# Autodesk Inventor assembly: Corpo_Interno
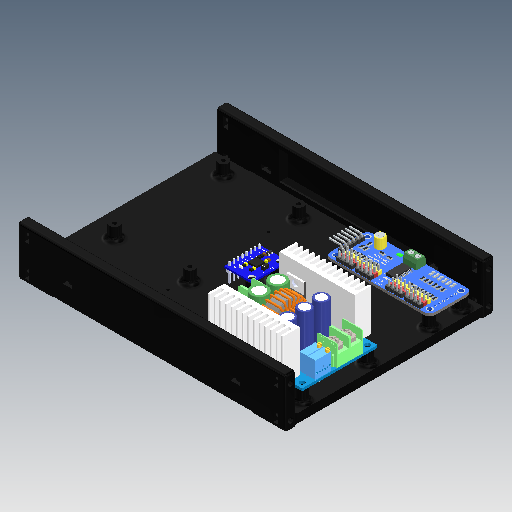
[picture p0: Inventor's stored thumbnail of the model, 512x512]
Saved by Autodesk Inventor 2020 (Build 240168000, 168)
## iProperties
Created: 2021-06-24
Part Number: Corpo_Interno
Document SubType Name: Assembly
Designer: JCarlos
Author: JCarlos
## Documents named in this file (7)
- C:\Users\candu\Google Drive\Doutorado_UTFPR\Projeto_1_SpotMicro\Projeto_3D\Robo_Montado_v3\3Dfiles_Q-Robot\Corpo_Interno_v3.iam
- C:\Users\candu\Google Drive\Doutorado_UTFPR\Projeto_1_SpotMicro\Projeto_3D\Robo_Montado_v3\3Dfiles_Q-Robot\Lateral.ipt
- C:\Users\candu\Google Drive\Doutorado_UTFPR\Projeto_1_SpotMicro\Projeto_3D\Robo_Montado_v3\3Dfiles_Q-Robot\StepDown\DC-DC Step Down Buck Converter CC-CV 300W 20A.iam
- C:\Users\candu\Google Drive\Doutorado_UTFPR\Projeto_1_SpotMicro\Projeto_3D\Robo_Montado_v3\3Dfiles_Q-Robot\Lateral_LadoUSB.ipt
- C:\Users\candu\Google Drive\Doutorado_UTFPR\Projeto_1_SpotMicro\Projeto_3D\Robo_Montado_v3\3Dfiles_Q-Robot\Base_Componentes_Arduino_v3.ipt
- C:\Users\candu\Google Drive\Doutorado_UTFPR\Projeto_1_SpotMicro\Projeto_3D\Robo_Montado_v3\3Dfiles_Q-Robot\DriverPCA9685\Arduino 16 Channel PWM Module\12Channel PWM.ipt
- C:\Users\candu\Google Drive\Doutorado_UTFPR\Projeto_1_SpotMicro\Projeto_3D\Robo_Montado_v3\3Dfiles_Q-Robot\Gyros\ITG-MPU.iam
## Components (6 placed, 6 different names)
1. Base_Componentes_Arduino_v3:1 — Coincidência:1, Coincidência:3, Coincidência:9, Coincidência:10, Ângulo:1, Coincidência:11, Coincidência:12, Ângulo:2, Coincidência:13, Coincidência:14, Ângulo:4, Coincidência:15, Coincidência:18, Alinhamento:1, Coincidência:19, Coincidência:20
2. Lateral:2 — Coincidência:1, Coincidência:3, Coincidência:15
3. 12Channel PWM:1 — Coincidência:10, Ângulo:1, Coincidência:11
4. ITG-MPU:1 [sub-assembly] — Coincidência:12, Ângulo:2, Coincidência:13
5. DC-DC Step Down Buck Converter CC-CV 300W 20A:1 [sub-assembly] — Coincidência:9, Coincidência:14, Ângulo:4
6. Lateral_LadoUSB:1 — Coincidência:18, Alinhamento:1, Coincidência:19
## Relationships (16: Mate 12, Angle 3, Flush 1)
- Coincidência:1 [Mate]: Base_Componentes_Arduino_v3:1 ↔ Lateral:2
- Coincidência:3 [Mate]: Base_Componentes_Arduino_v3:1 ↔ Lateral:2
- Coincidência:9 [Mate]: Base_Componentes_Arduino_v3:1 ↔ DC-DC Step Down Buck Converter CC-CV 300W 20A:1
- Coincidência:10 [Mate]: Base_Componentes_Arduino_v3:1 ↔ 12Channel PWM:1
- Ângulo:1 [Angle] (0 deg): Base_Componentes_Arduino_v3:1 ↔ 12Channel PWM:1
- Coincidência:11 [Mate]: Base_Componentes_Arduino_v3:1 ↔ 12Channel PWM:1
- Coincidência:12 [Mate]: Base_Componentes_Arduino_v3:1 ↔ ITG-MPU:1
- Ângulo:2 [Angle] (0 deg): Base_Componentes_Arduino_v3:1 ↔ ITG-MPU:1
- Coincidência:13 [Mate]: Base_Componentes_Arduino_v3:1 ↔ ITG-MPU:1
- Coincidência:14 [Mate]: Base_Componentes_Arduino_v3:1 ↔ DC-DC Step Down Buck Converter CC-CV 300W 20A:1
- Ângulo:4 [Angle] (0 deg): Base_Componentes_Arduino_v3:1 ↔ DC-DC Step Down Buck Converter CC-CV 300W 20A:1
- Coincidência:15 [Mate]: Base_Componentes_Arduino_v3:1 ↔ Lateral:2
- Coincidência:18 [Mate]: Base_Componentes_Arduino_v3:1 ↔ Lateral_LadoUSB:1
- Alinhamento:1 [Flush]: Base_Componentes_Arduino_v3:1 ↔ Lateral_LadoUSB:1
- Coincidência:19 [Mate]: Base_Componentes_Arduino_v3:1 ↔ Lateral_LadoUSB:1
- Coincidência:20 [Mate]: Base_Componentes_Arduino_v3:1
